# Autodesk Inventor assembly: hipjoint_toleg_left
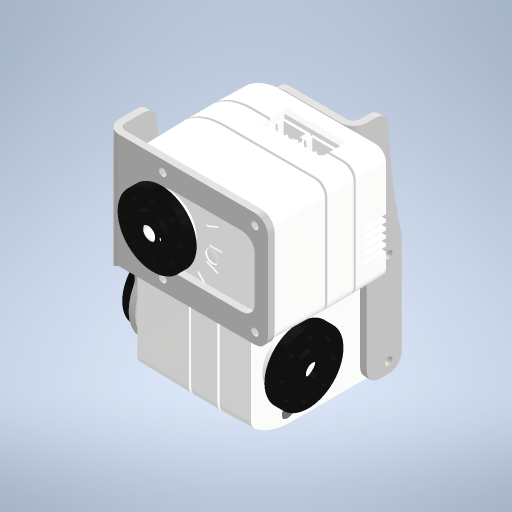
[picture p0: Inventor's stored thumbnail of the model, 512x512]
Saved by Autodesk Inventor 2024.1 (Build 281209000, 209)
## iProperties
Created: 2024-10-09
Part Number: hipjoint_toleg_left
Document SubType Name: Assembly
Designer: hibik
Author: hibik
## Documents named in this file (5)
- C:\Users\hibik\Documents\Robomech\HR\Eglantyne\hard\under_body\to_leg\hipjoint_toleg_left.iam
- C:\Users\hibik\Documents\Robomech\HR\Eglantyne\hard\needed_model\KRS3300モータ.ipt
- C:\Users\hibik\Documents\Robomech\HR\Eglantyne\hard\needed_model\KRS3300サーボホーン.ipt
- C:\Users\hibik\Documents\Robomech\HR\Eglantyne\hard\under_body\to_leg\hipjoint_toleg_under_left.ipt
- C:\Users\hibik\Documents\Robomech\HR\Eglantyne\hard\under_body\to_leg\hipjoint_toleg_upper_left.ipt
## Components (8 placed, 4 different names)
1. KRS3300モータ:1 — 挿入:4, 挿入:5, 挿入:8, 挿入:9, メイト:1
2. KRS3300モータ:2 — 挿入:6, 挿入:7, 挿入:10, 角度:1, 挿入:11
3. KRS3300サーボホーン:1 — 挿入:5
4. KRS3300サーボホーン:2 — 挿入:4
5. KRS3300サーボホーン:3 — 挿入:6
6. KRS3300サーボホーン:4 — 挿入:7
7. hipjoint_toleg_under_left:1 — 挿入:11, メイト:1
8. hipjoint_toleg_upper_left:1 — 挿入:8, 挿入:9, 挿入:10, 角度:1
## Relationships (10: Insert 8, Angle 1, Mate 1)
- 挿入:4 [Insert]: KRS3300モータ:1 ↔ KRS3300サーボホーン:2
- 挿入:5 [Insert]: KRS3300モータ:1 ↔ KRS3300サーボホーン:1
- 挿入:6 [Insert]: KRS3300モータ:2 ↔ KRS3300サーボホーン:3
- 挿入:7 [Insert]: KRS3300モータ:2 ↔ KRS3300サーボホーン:4
- 挿入:8 [Insert]: KRS3300モータ:1 ↔ hipjoint_toleg_upper_left:1
- 挿入:9 [Insert]: KRS3300モータ:1 ↔ hipjoint_toleg_upper_left:1
- 挿入:10 [Insert]: KRS3300モータ:2 ↔ hipjoint_toleg_upper_left:1
- 角度:1 [Angle] (0 deg): KRS3300モータ:2 ↔ hipjoint_toleg_upper_left:1
- 挿入:11 [Insert]: KRS3300モータ:2 ↔ hipjoint_toleg_under_left:1
- メイト:1 [Mate]: KRS3300モータ:1 ↔ hipjoint_toleg_under_left:1
